# Autodesk Inventor assembly: MXQ16-75A-M9B
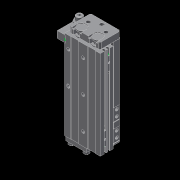
[picture p0: Inventor's stored thumbnail of the model, 180x180]
Saved by Autodesk Inventor 2021.1 (Build 251245000, 245)
## iProperties
Created: 2008-11-15
Part Number: MXQ16-75A-M9B
Document SubType Name: Assembly
変換規格: STEP AP214IS
ファイル名: MXMXQ161114192142281.step
プリプロセッサ: SolidWorks 2009
ポストプロセッサ: Build: 342, Release: 2008 SP3 - Date: Tue 05/27/2008
送信済み単位: MILLIMETERS
不明: 1e-05
Title: エアスライドテーブル
## Documents named in this file (7)
- Z:\inventorroom\sample\unit4\MXQ16-75A\MXQ16-75A-M9B.iam
- Z:\inventorroom\sample\unit4\MXQ16-75A\MXQ16-75A-M9B.step_ExtensionEnd_16A.iam
- Z:\inventorroom\sample\unit4\MXQ16-75A\MXQ16-75A-M9B.step_MXQTables_16-75.ipt
- Z:\inventorroom\sample\unit4\MXQ16-75A\MXQ16-75A-M9B.step_A9+F9_M9B.iam
- Z:\inventorroom\sample\unit4\MXQ16-75A\MXQ16-75A-M9B.step_TableMounting_16A.ipt
- Z:\inventorroom\sample\unit4\MXQ16-75A\MXQ16-75A-M9B.step_MXQ3149Tube_16-75.ipt
- Z:\inventorroom\sample\unit4\MXQ16-75A\MXQ16-75A-M9B.step_RetractionEnd_16A.iam
## Components (7 placed, 6 different names)
1. MXQ16-75A-M9B.step_ExtensionEnd_16A:1 [sub-assembly]
2. MXQ16-75A-M9B.step_MXQTables_16-75:1 — フラッシュ:1, フラッシュ:2, フラッシュ:3, フラッシュ:4, フラッシュ:5, 1
3. MXQ16-75A-M9B.step_A9+F9_M9B:1 [sub-assembly]
4. MXQ16-75A-M9B.step_TableMounting_16A:1 — フラッシュ:1, フラッシュ:2, フラッシュ:3
5. MXQ16-75A-M9B.step_A9+F9_M9B:2 [sub-assembly]
6. MXQ16-75A-M9B.step_MXQ3149Tube_16-75:1 — フラッシュ:4, フラッシュ:5, 1
7. MXQ16-75A-M9B.step_RetractionEnd_16A:1 [sub-assembly]
## Relationships (6: Flush 6)
- フラッシュ:1 [Flush] (0.2 mm): MXQ16-75A-M9B.step_MXQTables_16-75:1 ↔ MXQ16-75A-M9B.step_TableMounting_16A:1
- フラッシュ:2 [Flush] (14 mm): MXQ16-75A-M9B.step_MXQTables_16-75:1 ↔ MXQ16-75A-M9B.step_TableMounting_16A:1
- フラッシュ:3 [Flush] (103 mm): MXQ16-75A-M9B.step_MXQTables_16-75:1 ↔ MXQ16-75A-M9B.step_TableMounting_16A:1
- フラッシュ:4 [Flush] (5.5 mm): MXQ16-75A-M9B.step_MXQTables_16-75:1 ↔ MXQ16-75A-M9B.step_MXQ3149Tube_16-75:1
- フラッシュ:5 [Flush] (7 mm): MXQ16-75A-M9B.step_MXQTables_16-75:1 ↔ MXQ16-75A-M9B.step_MXQ3149Tube_16-75:1
- 1 [Flush] (1 mm): MXQ16-75A-M9B.step_MXQTables_16-75:1 ↔ MXQ16-75A-M9B.step_MXQ3149Tube_16-75:1
